# Autodesk Inventor assembly: HEAD_CAMERA_UNIT_ASM
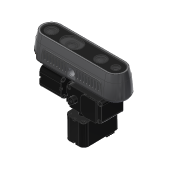
[picture p0: Inventor's stored thumbnail of the model, 180x180]
Saved by Autodesk Inventor 2019.4 (Build 234330000, 330)
## iProperties
Created: 2019-11-23
Part Number: HEAD_CAMERA_UNIT_ASM
Material: 一般
Document SubType Name: Assembly
Designer: y6tada
Author: y6tada
## Documents named in this file (4)
- C:\Workspace\Yuni9\Inventor\Asm\HEAD_CAMERA_UNIT\HEAD_CAMERA_UNIT_ASM.iam
- C:\Workspace\Yuni9\Inventor\Libs\Futaba RS30X\RS30x.ipt
- C:\Workspace\Yuni9\Inventor\Libs\Intel Realsense D435\Intel_RealSense_Depth_Camera_D435.iam
- C:\Workspace\Yuni9\Inventor\Libs\JAE Type C Conn\K3D-DX07VN24WA2-V2_JAE_Proprietary.ipt
## Components (5 placed, 3 different names)
1. RS30x:1
2. RS30x:2
3. RS30x:3
4. Intel_RealSense_Depth_Camera_D435:1 [sub-assembly]
5. K3D-DX07VN24WA2-V2_JAE_Proprietary:1
## Relationships (2: Mate 1, Flush 1)
- [Mate]: Intel_RealSense_Depth_Camera_D435:1 ↔ K3D-DX07VN24WA2-V2_JAE_Proprietary:1
- [Flush]: Intel_RealSense_Depth_Camera_D435:1 ↔ K3D-DX07VN24WA2-V2_JAE_Proprietary:1
